# Autodesk Inventor assembly: ASY PNS-Filter column D1200
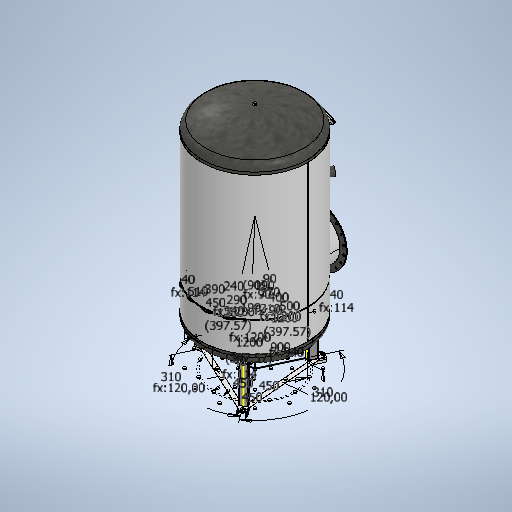
[picture p0: Inventor's stored thumbnail of the model, 512x512]
Saved by Autodesk Inventor 2025.1 (Build 291241020, 241B)
## iProperties
Created: 2025-02-13
Part Number: ASY PNS-Filter column D1200
Document SubType Name: Assembly
Designer: pokla
Mass: 522904 g
Surface Area: 229381 cm^2
Volume: 66871 cm^3
Density: 7.81959 g/cm^3
Author: pokla
Revision Number: 3
## iProperties of the stored document MemberDocs/xY4pnlgcvOs3ujohtUlbz05j1Wa
Created: 2025-02-13
Part Number: ASY PNS-Filter column D1200
Document SubType Name: Assembly
Designer: pokla
Mass: 522904 g
Surface Area: 229381 cm^2
Volume: 66871 cm^3
Density: 7.81959 g/cm^3
Author: pokla
Revision Number: 3
## iProperties of the stored document MemberDocs/xBqz0qcmpDsoxiitoCuizdwtuZb
Created: 2025-02-13
Part Number: ASY PNS-Filter column D1200
Document SubType Name: Assembly
Designer: pokla
Mass: 522904 g
Surface Area: 229381 cm^2
Volume: 66871 cm^3
Density: 7.81959 g/cm^3
Author: pokla
Revision Number: 3
## iProperties of the stored document MemberDocs/xTo33251kAkxzucsw5zkxq5ytLg
Created: 2025-02-13
Part Number: ASY PNS-Filter column D1200
Document SubType Name: Assembly
Designer: pokla
Mass: 522904 g
Surface Area: 229381 cm^2
Volume: 66871 cm^3
Density: 7.81959 g/cm^3
Author: pokla
Revision Number: 3
## iProperties of the stored document MemberDocs/xZox4hcbvPckmhach2bc1j5mcOh
Created: 2025-02-13
Part Number: ASY PNS-Filter column D1200
Document SubType Name: Assembly
Designer: pokla
Mass: 522904 g
Surface Area: 229381 cm^2
Volume: 66871 cm^3
Density: 7.81959 g/cm^3
Author: pokla
Revision Number: 3
## Documents named in this file (48)
- C:\Users\admin\Yandex.Disk\home pc\Inventor\PNS2-Panaevsk\Filter D1200\ASY PNS-Filter column D1200.iam
- C:\Users\user\YandexDisk-badmisterfox\home pc\Inventor\PNS-Panaevsk\Filter D1200\PNS-712 accses hatch flangeipt.ipt
- C:\Users\user\YandexDisk-badmisterfox\home pc\Inventor\PNS-Panaevsk\Filter D1200\000 DIM PNS-Filter column D1200.ipt
- C:\Users\user\YandexDisk-badmisterfox\home pc\Inventor\PNS-Panaevsk\Filter D1200\PNS-711 accses hatch tube.ipt
- C:\Users\user\YandexDisk-badmisterfox\home pc\Inventor\PNS-Panaevsk\Filter D1200\PNS-701 main tube D1200.ipt
- C:\Users\user\YandexDisk-badmisterfox\home pc\Inventor\PNS-Panaevsk\Filter D1200\PNS- 752 tube.ipt
- C:\Users\user\YandexDisk-badmisterfox\home pc\Inventor\PNS-Panaevsk\Filter D1200\PNV - 704 dished head D1200.ipt
- C:\Users\user\YandexDisk-badmisterfox\home pc\Inventor\PNS-Panaevsk\Filter D1200\Fitting G1.ipt
- C:\Users\user\YandexDisk-badmisterfox\home pc\Inventor\PNS-Panaevsk\Filter D1200\PNS- 723 charging half tube.ipt
- C:\Users\user\YandexDisk-badmisterfox\home pc\Inventor\PNS-Panaevsk\CC\en-US\DIN 2576 PN 10(2)\DIN 2576 Slip-On Flange for Welding Series 1 (ISO) - PN 10 500 x 508.ipt
- C:\Users\user\YandexDisk-badmisterfox\home pc\Inventor\PNS-Panaevsk\Filter D1200\ASY PNS780-Filter legs D1200.iam
- C:\Users\user\YandexDisk-badmisterfox\home pc\Inventor\PNS-Panaevsk\Filter D1000\DIN 2576 Slip-On Flange for Welding Series 1 (ISO) - PN 10 80 x 88.9.ipt
- C:\Users\user\YandexDisk-badmisterfox\home pc\Inventor\PNS-Panaevsk\Filter D1200\PNS-733 charging flange round.ipt
- C:\Users\user\YandexDisk-badmisterfox\home pc\Inventor\PNS-Panaevsk\Filter D1200\sprinkler dummy.ipt
- C:\Users\user\YandexDisk-badmisterfox\home pc\Inventor\PNS-Panaevsk\CC\en-US\DIN 2615-1 T\DIN 2615-1 Tee 88.9 x 5.6 S.ipt
- C:\Users\user\YandexDisk-badmisterfox\home pc\Inventor\PNS-Panaevsk\CC\en-US\DIN 2616 CR (K)\DIN 2616 Concentric Reducer (K) 88.9 x 2.3 - 48.3 x 2.ipt
- C:\Users\user\YandexDisk-badmisterfox\home pc\Inventor\PNS-Panaevsk\Filter D1000\ASY PNS-722 charging hatch.iam
- C:\Users\user\YandexDisk-badmisterfox\home pc\Inventor\PNS-Panaevsk\Filter D1200\PNS-734 charging flange cup.ipt
- C:\Users\user\YandexDisk-badmisterfox\home pc\Inventor\PNS-Panaevsk\Filter D1200\PNS 753 FDS tube.ipt
- C:\Users\user\YandexDisk-badmisterfox\home pc\Inventor\PNS-Panaevsk\Filter D1200\ASY PNS 741 bottom FDS1 D1200.iam
- C:\Users\user\YandexDisk-badmisterfox\home pc\Inventor\PNS-Panaevsk\CC\en-US\JIS B 2312 90 (2)\JIS B 2312 90 Deg Long Elbow Steel 80A x Sch 40.ipt
- C:\Users\user\YandexDisk-badmisterfox\home pc\Inventor\PNS-Panaevsk\Workspace\ASY PNS 750 filter-distribution-system 1200.iam
- C:\Users\user\YandexDisk-badmisterfox\home pc\Inventor\PNS-Panaevsk\Filter D1200\PNS 755 FDS tube.ipt
- C:\Users\user\YandexDisk-badmisterfox\home pc\Inventor\PNS-Panaevsk\Filter D1200\PNS 734 FDS flange DN90.ipt
- C:\Users\user\YandexDisk-badmisterfox\home pc\Inventor\PNS-Panaevsk\Filter D1200\PNS 735 FDS free flange DN90.ipt
- C:\Users\user\YandexDisk-badmisterfox\home pc\Inventor\PNS-Panaevsk\Filter D1200\PNS 756 FDS tube.ipt
- C:\Users\admin\Yandex.Disk\home pc\Inventor\PNS2-Panaevsk\Filter D1200\PNS-712 accses hatch flangeipt.ipt
- C:\Users\admin\Yandex.Disk\home pc\Inventor\PNS2-Panaevsk\Filter D1200\000 DIM PNS-Filter column D1200.ipt
- C:\Users\admin\Yandex.Disk\home pc\Inventor\PNS2-Panaevsk\Filter D1200\PNS-711 accses hatch tube.ipt
- C:\Users\admin\Yandex.Disk\home pc\Inventor\PNS2-Panaevsk\Filter D1200\PNS-701 main tube D1200.ipt
- C:\Users\admin\Yandex.Disk\home pc\Inventor\PNS2-Panaevsk\Filter D1200\PNS- 752 tube.ipt
- C:\Users\admin\Yandex.Disk\home pc\Inventor\PNS2-Panaevsk\Filter D1200\PNV - 704 dished head D1200.ipt
- C:\Users\admin\Yandex.Disk\home pc\Inventor\PNS2-Panaevsk\Filter D1200\Fitting G1.ipt
- C:\Users\admin\Yandex.Disk\home pc\Inventor\PNS2-Panaevsk\Filter D1200\PNS- 723 charging half tube.ipt
- C:\Users\admin\Yandex.Disk\home pc\Inventor\PNS2-Panaevsk\CC\en-US\DIN 2576 PN 10(2)\DIN 2576 Slip-On Flange for Welding Series 1 (ISO) - PN 10 500 x 508.ipt
- C:\Users\admin\Yandex.Disk\home pc\Inventor\PNS2-Panaevsk\Filter D1200\ASY PNS780-Filter legs D1200.iam
- C:\Users\admin\Yandex.Disk\home pc\Inventor\PNS2-Panaevsk\Filter D1000\DIN 2576 Slip-On Flange for Welding Series 1 (ISO) - PN 10 80 x 88.9.ipt
- C:\Users\admin\Yandex.Disk\home pc\Inventor\PNS2-Panaevsk\Filter D1200\PNS-733 charging flange round.ipt
- C:\Users\admin\Yandex.Disk\home pc\Inventor\PNS2-Panaevsk\Filter D1200\sprinkler dummy.ipt
- C:\Users\admin\Yandex.Disk\home pc\Inventor\PNS2-Panaevsk\CC\en-US\DIN 2615-1 T\DIN 2615-1 Tee 88.9 x 5.6 S.ipt
- C:\Users\admin\Yandex.Disk\home pc\Inventor\PNS2-Panaevsk\CC\en-US\DIN 2616 CR (K)\DIN 2616 Concentric Reducer (K) 88.9 x 2.3 - 48.3 x 2.ipt
- C:\Users\admin\Yandex.Disk\home pc\Inventor\PNS2-Panaevsk\Filter D1000\ASY PNS-722 charging hatch.iam
- C:\Users\admin\Yandex.Disk\home pc\Inventor\PNS2-Panaevsk\Filter D1200\PNS-734 charging flange cup.ipt
- C:\Users\admin\Yandex.Disk\home pc\Inventor\PNS2-Panaevsk\Filter D1200\PNS 753 FDS tube.ipt
- C:\Users\admin\Yandex.Disk\home pc\Inventor\PNS2-Panaevsk\Filter D1200\ASY PNS 741 bottom FDS1 D1200.iam
- C:\Users\admin\Yandex.Disk\home pc\Inventor\PNS2-Panaevsk\CC\en-US\JIS B 2312 90 (2)\JIS B 2312 90 Deg Long Elbow Steel 80A x Sch 40.ipt
- C:\Users\admin\Yandex.Disk\home pc\Inventor\PNS2-Panaevsk\filter-distribution-system\ASY PNS 750 filter-distribution-system 1200.iam
- C:\Users\admin\Yandex.Disk\home pc\Inventor\PNS2-Panaevsk\Filter D1200\ASY PNS 760 elbow.iam
## Components (76 placed, 25 different names)
1. 000 DIM PNS-Filter column D1200.ipt:1
2. PNS-711 accses hatch tube.ipt:1 — Rigid:10, Rigid:50
3. PNS-701 main tube D1200.ipt:1 — Rigid:10, Rigid:13, Rigid:14, Mate:1, Mate:2, Rigid:33, Rigid:36, Rigid:52, Rigid:64
4. PNV - 704 dished head D1200.ipt:1 — Rigid:13, Rigid:16
5. PNV - 704 dished head D1200.ipt:2 — Rigid:14, Rigid:15, Mate:3
6. Fitting G1.ipt:1 — Rigid:15
7. Fitting G1.ipt:2 — Rigid:16
8. PNS- 723 charging half tube.ipt:2 — Rigid:32, Rigid:33, Rigid:36
9. DIN 2576 Slip-On Flange for Welding Series 1 (ISO) - PN 10 500 x 508.ipt:1
10. PNS-712 accses hatch flangeipt.ipt:3 — Rotational:4, Rigid:50
11. Assembly2.iam:1 [sub-assembly] — Flush:2, Mate:4, Angle:1
12. PNS-733 charging flange round:1 — Rigid:32, Rigid:51
13. DIN 2576 Slip-On Flange for Welding Series 1 (ISO) - PN 10 80 x 88.9:2
14. DIN 2615-1 Tee 88.9 x 5.6 S:2 — Rigid:46, Rigid:48, Rigid:53
15. Труба подключения фильтра D1200:5
16. DIN 2616 Concentric Reducer (K) 88.9 x 2.3 - 48.3 x 2:2
17. DIN 2616 Concentric Reducer (K) 88.9 x 2.3 - 48.3 x 2:3 — Rigid:46
18. DIN 2616 Concentric Reducer (K) 88.9 x 2.3 - 48.3 x 2:4
19. DIN 2616 Concentric Reducer (K) 88.9 x 2.3 - 48.3 x 2:5 — Rigid:48
20. DIN 2616 Concentric Reducer (K) 88.9 x 2.3 - 48.3 x 2:6
21. ASY PNS-722 charging hatch:1 [sub-assembly] — Rotational:4
22. PNS-734 charging flange cup:1 — Rigid:51
23. PNS 753 FDS tube:1 — Rigid:53, Rigid:54, Rigid:64
24. ASY PNS 741 bottom FDS1 D1200:1 [sub-assembly] — Rigid:52, Rigid:63
25. JIS B 2312 90 Deg Long Elbow Steel 80A x Sch 40:1 — Rigid:54, Rigid:55
26. JIS B 2312 90 Deg Long Elbow Steel 80A x Sch 40:2 — Rigid:59, Rigid:60
27. ASY PNS 750 filter-distribution-system 1200:1 [sub-assembly] — Rotational:5, Angle:2
28. Труба подключения фильтра D1200:6 — Rigid:55, Rigid:56
29. DIN 2576 Slip-On Flange for Welding Series 1 (ISO) - PN 10 80 x 88.9:3 — Rigid:56
30. PNS 755 FDS tube:1 — Rigid:57, Rigid:58, Rigid:59
31. PNS 734 FDS flange DN90:1 — Rigid:58
32. PNS 735 FDS free flange DN90:1 — Rigid:57, Rigid:63
33. PNS 756 FDS tube:1 — Rigid:60, Rigid:61
34. PNS 734 FDS flange DN90:2 — Rigid:62, Rotational:5
35. PNS 735 FDS free flange DN90:2 — Rigid:61, Rigid:62
36. sprinkler dummy:1
37. sprinkler dummy:2
38. sprinkler dummy:3
39. sprinkler dummy:4
40. sprinkler dummy:5
41. sprinkler dummy:6
42. sprinkler dummy:7
43. sprinkler dummy:8
44. sprinkler dummy:9
45. sprinkler dummy:10
46. sprinkler dummy:11
47. sprinkler dummy:12
48. sprinkler dummy:13
49. sprinkler dummy:14
50. sprinkler dummy:15
51. sprinkler dummy:16
52. sprinkler dummy:17
53. sprinkler dummy:18
54. sprinkler dummy:19
55. sprinkler dummy:20
56. sprinkler dummy:21
57. sprinkler dummy:22
58. sprinkler dummy:23
59. sprinkler dummy:24
60. sprinkler dummy:25
61. sprinkler dummy:26
62. sprinkler dummy:27
63. sprinkler dummy:28
64. sprinkler dummy:29
65. sprinkler dummy:30
66. sprinkler dummy:31
67. sprinkler dummy:32
68. sprinkler dummy:33
69. sprinkler dummy:34
70. sprinkler dummy:35
71. sprinkler dummy:36
72. sprinkler dummy:37
73. sprinkler dummy:38
74. sprinkler dummy:39
75. sprinkler dummy:40
76. sprinkler dummy:41
## Relationships (39: WeldJoint 29, Mate 4, RevoluteJoint 3, Angle 2, Flush 1)
- Rigid:10 [WeldJoint] (100 mm): PNS-711 accses hatch tube.ipt:1 ↔ PNS-701 main tube D1200.ipt:1
- Rigid:13 [WeldJoint]: PNS-701 main tube D1200.ipt:1 ↔ PNV - 704 dished head D1200.ipt:1
- Rigid:14 [WeldJoint]: PNS-701 main tube D1200.ipt:1 ↔ PNV - 704 dished head D1200.ipt:2
- Rigid:15 [WeldJoint]: PNV - 704 dished head D1200.ipt:2 ↔ Fitting G1.ipt:1
- Rigid:16 [WeldJoint]: PNV - 704 dished head D1200.ipt:1 ↔ Fitting G1.ipt:2
- Mate:1: PNS-701 main tube D1200.ipt:1
- Mate:2: PNS-701 main tube D1200.ipt:1
- Mate:3 (2610 mm): PNV - 704 dished head D1200.ipt:2
- Flush:2: Assembly2.iam:1
- Rigid:32 [WeldJoint]: PNS- 723 charging half tube.ipt:2 ↔ PNS-733 charging flange round:1
- Mate:4: Assembly2.iam:1
- Angle:1 (145 deg): Assembly2.iam:1
- Rigid:33 [WeldJoint]: PNS-701 main tube D1200.ipt:1 ↔ PNS- 723 charging half tube.ipt:2
- Rigid:36 [WeldJoint]: PNS-701 main tube D1200.ipt:1 ↔ PNS- 723 charging half tube.ipt:2
- [RevoluteJoint]: DIN 2615-1 Tee 88.9 x 5.6 S:2 ↔ Труба подключения фильтра D1200:5
- [WeldJoint]: DIN 2576 Slip-On Flange for Welding Series 1 (ISO) - PN 10 80 x 88.9:2 ↔ Труба подключения фильтра D1200:5
- [WeldJoint]: DIN 2615-1 Tee 88.9 x 5.6 S:2 ↔ DIN 2616 Concentric Reducer (K) 88.9 x 2.3 - 48.3 x 2:2
- Rigid:46 [WeldJoint]: DIN 2615-1 Tee 88.9 x 5.6 S:2 ↔ DIN 2616 Concentric Reducer (K) 88.9 x 2.3 - 48.3 x 2:3
- [WeldJoint]: DIN 2616 Concentric Reducer (K) 88.9 x 2.3 - 48.3 x 2:4 ↔ ASY PNS 741 bottom FDS1 D1200:1
- Rigid:48 [WeldJoint]: DIN 2615-1 Tee 88.9 x 5.6 S:2 ↔ DIN 2616 Concentric Reducer (K) 88.9 x 2.3 - 48.3 x 2:5
- [WeldJoint]: DIN 2616 Concentric Reducer (K) 88.9 x 2.3 - 48.3 x 2:6 ↔ ASY PNS 741 bottom FDS1 D1200:1
- Rotational:4 [RevoluteJoint]: PNS-712 accses hatch flangeipt.ipt:3 ↔ ASY PNS-722 charging hatch:1
- Rigid:50 [WeldJoint]: PNS-711 accses hatch tube.ipt:1 ↔ PNS-712 accses hatch flangeipt.ipt:3
- Rigid:51 [WeldJoint]: PNS-733 charging flange round:1 ↔ PNS-734 charging flange cup:1
- Rigid:52 [WeldJoint] (43 mm): PNS-701 main tube D1200.ipt:1 ↔ ASY PNS 741 bottom FDS1 D1200:1
- Rigid:53 [WeldJoint]: DIN 2615-1 Tee 88.9 x 5.6 S:2 ↔ PNS 753 FDS tube:1
- Rigid:54 [WeldJoint]: PNS 753 FDS tube:1 ↔ JIS B 2312 90 Deg Long Elbow Steel 80A x Sch 40:1
- Rigid:55 [WeldJoint]: JIS B 2312 90 Deg Long Elbow Steel 80A x Sch 40:1 ↔ Труба подключения фильтра D1200:6
- Rigid:56 [WeldJoint]: Труба подключения фильтра D1200:6 ↔ DIN 2576 Slip-On Flange for Welding Series 1 (ISO) - PN 10 80 x 88.9:3
- Rigid:57 [WeldJoint]: PNS 755 FDS tube:1 ↔ PNS 735 FDS free flange DN90:1
- Rigid:58 [WeldJoint]: PNS 755 FDS tube:1 ↔ PNS 734 FDS flange DN90:1
- Rigid:59 [WeldJoint]: JIS B 2312 90 Deg Long Elbow Steel 80A x Sch 40:2 ↔ PNS 755 FDS tube:1
- Rigid:60 [WeldJoint]: JIS B 2312 90 Deg Long Elbow Steel 80A x Sch 40:2 ↔ PNS 756 FDS tube:1
- Rigid:61 [WeldJoint]: PNS 756 FDS tube:1 ↔ PNS 735 FDS free flange DN90:2
- Rigid:62 [WeldJoint]: PNS 734 FDS flange DN90:2 ↔ PNS 735 FDS free flange DN90:2
- Rigid:63 [WeldJoint]: ASY PNS 741 bottom FDS1 D1200:1 ↔ PNS 735 FDS free flange DN90:1
- Rigid:64 [WeldJoint] (45 mm): PNS-701 main tube D1200.ipt:1 ↔ PNS 753 FDS tube:1
- Rotational:5 [RevoluteJoint]: ASY PNS 750 filter-distribution-system 1200:1 ↔ PNS 734 FDS flange DN90:2
- Angle:2 (180 deg): ASY PNS 750 filter-distribution-system 1200:1
## Named parameters: d74_d69 = 0 mm, d75_d70 = 110 deg, d76_d71 = 0 mm, d77_d72 = 0 mm
